# Autodesk Inventor assembly: Blue Alliance Bucket
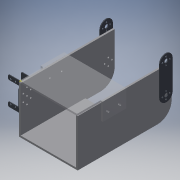
[picture p0: Inventor's stored thumbnail of the model, 180x180]
Saved by Autodesk Inventor 2016 (Build 200138000, 138)
## iProperties
Created: 2015-12-16
Part Number: Blue Alliance Bucket
Document SubType Name: Assembly
Designer: TimB
Author: TimB
## Documents named in this file (5)
- C:\Users\TimB\Documents\GitHub\phi_robotics\3d-models\FTC_Tetrix_KOP_Block_Party\Tim Bloot Designs\JAr JaR Bot\Blue Alliance Bucket.iam
- C:\Users\TimB\Documents\GitHub\phi_robotics\3d-models\FTC_Tetrix_KOP_Block_Party\Tim Bloot Designs\JAr JaR Bot\Bucket - BlueA.ipt
- C:\Users\TimB\Documents\GitHub\phi_robotics\3d-models\FTC_Tetrix_KOP_Block_Party\Tetrix_Kit_FTC\Autodesk Inventor Files\tetrix_servo_mount.ipt
- C:\Users\TimB\Documents\GitHub\phi_robotics\3d-models\FTC_Tetrix_KOP_Block_Party\Tetrix_Kit_FTC\Autodesk Inventor Files\tetrix_739061_2012.ipt
- C:\Users\TimB\Documents\GitHub\phi_robotics\3d-models\FTC_Tetrix_KOP_Block_Party\Tim Bloot Designs\JAr JaR Bot\Bucket -  Top.ipt
## Components (5 placed, 4 different names)
1. Bucket - BlueA:1 — Rigid:1, Rigid:2, Rigid:3, Rigid:4
2. tetrix_servo_mount:1 — Rigid:1
3. tetrix_739061_2012:1 — Rigid:2
4. tetrix_739061_2012:2 — Rigid:3
5. Bucket -  Top:1 — Rigid:4
## Relationships (4: WeldJoint 4)
- Rigid:1 [WeldJoint]: Bucket - BlueA:1 ↔ tetrix_servo_mount:1
- Rigid:2 [WeldJoint]: Bucket - BlueA:1 ↔ tetrix_739061_2012:1
- Rigid:3 [WeldJoint]: Bucket - BlueA:1 ↔ tetrix_739061_2012:2
- Rigid:4 [WeldJoint]: Bucket - BlueA:1 ↔ Bucket -  Top:1
